# Autodesk Inventor assembly: Cabin Wall Assembly
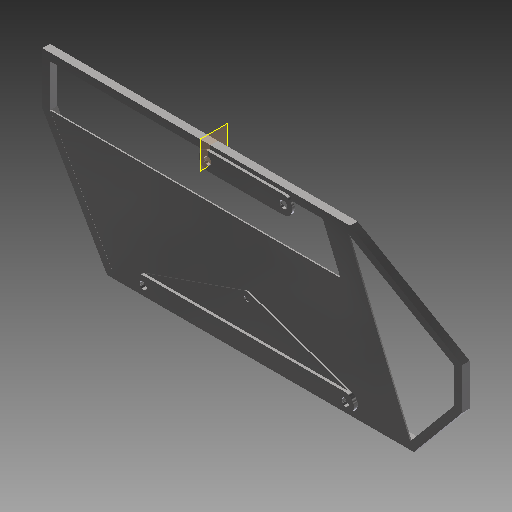
[picture p0: Inventor's stored thumbnail of the model, 512x512]
Saved by Autodesk Inventor 2019 (Build 230136000, 136)
## iProperties
Created: 2019-08-30
Part Number: Cabin Wall Assembly
Document SubType Name: Assembly
Designer: DIBYOJYOTI
Author: DIBYOJYOTI
## Documents named in this file (4)
- D:\Autocad\Cabin Wall Assembly.iam
- D:\Autocad\Cabin Frame.ipt
- D:\Autocad\Cabin Side Panel.ipt
- D:\Autocad\Cabin Hold.ipt
## Components (3 placed, 3 different names)
1. Cabin Frame:1 — Flush:1, Flush:3
2. Cabin Side Panel:1 — Flush:1, Flush:2
3. Cabin Hold:1 — Flush:2, Flush:3
## Relationships (3: Flush 3)
- Flush:1: Cabin Frame:1 ↔ Cabin Side Panel:1
- Flush:2 (-1 mm): Cabin Side Panel:1 ↔ Cabin Hold:1
- Flush:3 (3 mm): Cabin Frame:1 ↔ Cabin Hold:1
